# Autodesk Inventor assembly: InkrementalisFoliaEsNullAtmenet
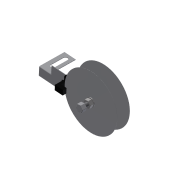
[picture p0: Inventor's stored thumbnail of the model, 180x180]
Saved by Autodesk Inventor 2015 SP1 (Build 190203100, 203)
## iProperties
Created: 2015-02-26
Part Number: InkrementalisFoliaEsNullAtmenet
Document SubType Name: Assembly
Designer: laca
Author: laca
## Documents named in this file (7)
- C:\Users\laca\Desktop\Allamvizsga\Invntor\RobotMechanikaForMAtlabVer2\InkrementalisFoliaEsNullAtmenet.iam
- C:\Users\laca\Desktop\Allamvizsga\Invntor\RobotMechanikaForMAtlabVer2\SzenzorCsavar5os.ipt
- C:\Users\laca\Desktop\Allamvizsga\Invntor\RobotMechanikaForMAtlabVer2\JIS B 1181 - M5(1).ipt
- C:\Users\laca\Desktop\Allamvizsga\Invntor\RobotMechanikaForMAtlabVer2\ISO 7089 - 5 - 140 HV(1).ipt
- C:\Users\laca\Desktop\Allamvizsga\Invntor\RobotMechanikaForMAtlabVer2\InkrementalisFolia.ipt
- C:\Users\laca\Desktop\Allamvizsga\Invntor\RobotMechanikaForMAtlabVer2\InkrementalisOptikaiErzekelo.ipt
- C:\Users\laca\Desktop\Allamvizsga\Invntor\RobotMechanikaForMAtlabVer2\SenzorTarto.ipt
## Components (14 placed, 6 different names)
1. SzenzorCsavar5os:1 — Mate:5
2. JIS B 1181 finished Class 2 - Metric Class 2 finished M5:1 — Mate:5
3. JIS B 1181 finished Class 2 - Metric Class 2 finished M5:2
4. ISO 7089 5 - 140 HV:1
5. ISO 7089 5 - 140 HV:2
6. ISO 7089 5 - 140 HV:3
7. ISO 7089 5 - 140 HV:4
8. JIS B 1181 finished Class 2 - Metric Class 2 finished M5:3
9. JIS B 1181 finished Class 2 - Metric Class 2 finished M5:4
10. InkrementalisFolia:1 — Mate:3
11. InkrementalisFolia:2
12. InkrementalisOptikaiErzekelo:1 — Mate:3, Insert:9, Insert:10, Mate:4
13. InkrementalisOptikaiErzekelo:2 — Insert:9, Insert:10, Insert:11
14. SenzorTarto:1 — Insert:11, Mate:4
## Relationships (18: Insert 11, Mate 5, CylindricalJoint 2)
- [CylindricalJoint]: SzenzorCsavar5os:1 ↔ JIS B 1181 finished Class 2 - Metric Class 2 finished M5:1
- [Mate]: SzenzorCsavar5os:1 ↔ JIS B 1181 finished Class 2 - Metric Class 2 finished M5:1
- [Insert]: JIS B 1181 finished Class 2 - Metric Class 2 finished M5:1 ↔ ISO 7089 5 - 140 HV:1
- [Insert]: JIS B 1181 finished Class 2 - Metric Class 2 finished M5:2 ↔ ISO 7089 5 - 140 HV:4
- [CylindricalJoint]: SzenzorCsavar5os:1 ↔ JIS B 1181 finished Class 2 - Metric Class 2 finished M5:4
- [Insert]: ISO 7089 5 - 140 HV:2 ↔ JIS B 1181 finished Class 2 - Metric Class 2 finished M5:4
- [Insert]: ISO 7089 5 - 140 HV:3 ↔ JIS B 1181 finished Class 2 - Metric Class 2 finished M5:3
- [Insert]: ISO 7089 5 - 140 HV:1 ↔ InkrementalisFolia:2
- [Insert]: ISO 7089 5 - 140 HV:2 ↔ InkrementalisFolia:1
- [Mate] (15 mm): InkrementalisFolia:1 ↔ InkrementalisFolia:2
- [Insert]: ISO 7089 5 - 140 HV:2 ↔ ISO 7089 5 - 140 HV:4
- [Insert]: ISO 7089 5 - 140 HV:1 ↔ ISO 7089 5 - 140 HV:3
- Mate:3 (2 mm): InkrementalisFolia:1 ↔ InkrementalisOptikaiErzekelo:1
- Insert:9 (2 mm): InkrementalisOptikaiErzekelo:1 ↔ InkrementalisOptikaiErzekelo:2
- Insert:10: InkrementalisOptikaiErzekelo:1 ↔ InkrementalisOptikaiErzekelo:2
- Insert:11: InkrementalisOptikaiErzekelo:2 ↔ SenzorTarto:1
- Mate:4: InkrementalisOptikaiErzekelo:1 ↔ SenzorTarto:1
- Mate:5 (4 mm): SzenzorCsavar5os:1 ↔ JIS B 1181 finished Class 2 - Metric Class 2 finished M5:1
